# Autodesk Inventor assembly: camaravision
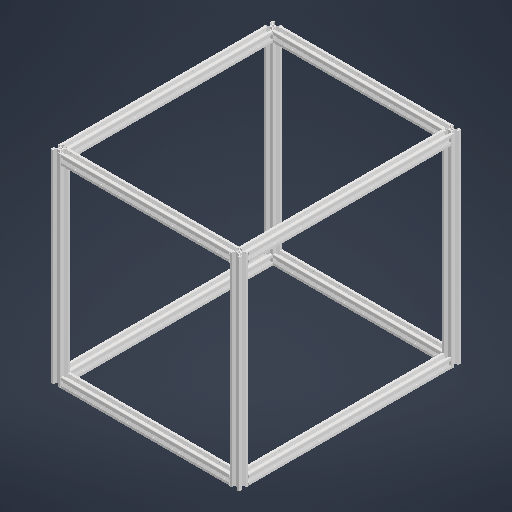
[picture p0: Inventor's stored thumbnail of the model, 512x512]
Saved by Autodesk Inventor 2026.2 (Build 302298010, 298A)
## iProperties
Created: 2026-04-14
Part Number: camaravision
Document SubType Name: Assembly
Designer: grego
Author: grego
## Documents named in this file (4)
- C:\Users\grego\OneDrive\Escritorio\PDM\camaravision.iam
- C:\Users\grego\OneDrive\Escritorio\PDM\VSLOT20x20x400.ipt
- C:\Users\grego\OneDrive\Escritorio\PDM\VSLOT20x20x420.ipt
- C:\Users\grego\OneDrive\Escritorio\PDM\VSLOT20x20x350.ipt
## Components (12 placed, 3 different names)
1. VSLOT20x20x400:1 — Mate:1, Flush:1, Flush:2, Mate:5, Flush:9, Flush:10, Mate:6, Flush:11, Flush:12
2. VSLOT20x20x420:1 — Mate:1, Flush:1, Flush:2, Mate:2, Flush:3, Flush:4
3. VSLOT20x20x400:2 — Mate:2, Flush:3, Flush:4, Mate:3, Flush:5, Flush:6, Mate:4, Flush:7, Flush:8, Mate:7, Flush:13, Flush:14
4. VSLOT20x20x420:2 — Mate:3, Flush:5, Flush:6
5. VSLOT20x20x350:1 — Mate:4, Flush:7, Flush:8
6. VSLOT20x20x350:2 — Mate:7, Flush:13, Flush:14, Mate:8, Mate:9, Flush:15, Flush:16
7. VSLOT20x20x350:3 — Mate:6, Flush:11, Flush:12, Mate:10, Flush:17, Flush:18
8. VSLOT20x20x350:4 — Mate:5, Flush:9, Flush:10
9. VSLOT20x20x420:3 — Mate:10, Flush:17, Flush:18, Mate:11, Flush:19, Flush:20, Mate:12, Flush:21, Flush:22
10. VSLOT20x20x420:4 — Mate:8, Mate:9, Flush:15, Flush:16
11. VSLOT20x20x400:3 — Mate:11, Flush:19, Flush:20
12. VSLOT20x20x400:4 — Mate:12, Flush:21, Flush:22
## Relationships (34: Flush 22, Mate 12)
- Mate:1: VSLOT20x20x400:1 ↔ VSLOT20x20x420:1
- Flush:1: VSLOT20x20x400:1 ↔ VSLOT20x20x420:1
- Flush:2: VSLOT20x20x400:1 ↔ VSLOT20x20x420:1
- Mate:2: VSLOT20x20x420:1 ↔ VSLOT20x20x400:2
- Flush:3: VSLOT20x20x420:1 ↔ VSLOT20x20x400:2
- Flush:4: VSLOT20x20x420:1 ↔ VSLOT20x20x400:2
- Mate:3: VSLOT20x20x400:2 ↔ VSLOT20x20x420:2
- Flush:5: VSLOT20x20x400:2 ↔ VSLOT20x20x420:2
- Flush:6: VSLOT20x20x400:2 ↔ VSLOT20x20x420:2
- Mate:4: VSLOT20x20x400:2 ↔ VSLOT20x20x350:1
- Flush:7: VSLOT20x20x400:2 ↔ VSLOT20x20x350:1
- Flush:8: VSLOT20x20x400:2 ↔ VSLOT20x20x350:1
- Mate:5: VSLOT20x20x400:1 ↔ VSLOT20x20x350:4
- Flush:9: VSLOT20x20x400:1 ↔ VSLOT20x20x350:4
- Flush:10: VSLOT20x20x400:1 ↔ VSLOT20x20x350:4
- Mate:6: VSLOT20x20x400:1 ↔ VSLOT20x20x350:3
- Flush:11: VSLOT20x20x400:1 ↔ VSLOT20x20x350:3
- Flush:12: VSLOT20x20x400:1 ↔ VSLOT20x20x350:3
- Mate:7: VSLOT20x20x400:2 ↔ VSLOT20x20x350:2
- Flush:13: VSLOT20x20x400:2 ↔ VSLOT20x20x350:2
- Flush:14: VSLOT20x20x400:2 ↔ VSLOT20x20x350:2
- Mate:8: VSLOT20x20x350:2 ↔ VSLOT20x20x420:4
- Mate:9: VSLOT20x20x350:2 ↔ VSLOT20x20x420:4
- Flush:15: VSLOT20x20x350:2 ↔ VSLOT20x20x420:4
- Flush:16: VSLOT20x20x350:2 ↔ VSLOT20x20x420:4
- Mate:10: VSLOT20x20x350:3 ↔ VSLOT20x20x420:3
- Flush:17: VSLOT20x20x350:3 ↔ VSLOT20x20x420:3
- Flush:18: VSLOT20x20x350:3 ↔ VSLOT20x20x420:3
- Mate:11: VSLOT20x20x420:3 ↔ VSLOT20x20x400:3
- Flush:19: VSLOT20x20x420:3 ↔ VSLOT20x20x400:3
- Flush:20: VSLOT20x20x420:3 ↔ VSLOT20x20x400:3
- Mate:12: VSLOT20x20x420:3 ↔ VSLOT20x20x400:4
- Flush:21: VSLOT20x20x420:3 ↔ VSLOT20x20x400:4
- Flush:22: VSLOT20x20x420:3 ↔ VSLOT20x20x400:4
